# Autodesk Inventor assembly: ASY ДМФ 0100 Барабан v2.1
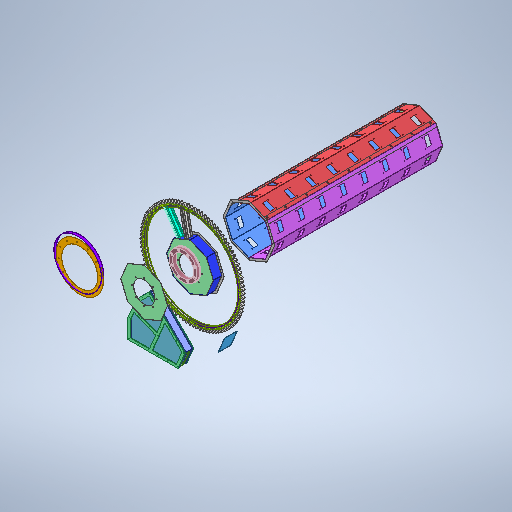
[picture p0: Inventor's stored thumbnail of the model, 512x512]
Saved by Autodesk Inventor 2025 (Build 290162010, 162A)
## iProperties
Created: 2024-04-28
Part Number: ASY ДМФ 0100 Барабан v2.1
Document SubType Name: Assembly
Designer: pokla
Author: pokla
## Documents named in this file (23)
- C:\Users\pokla\Documents\Inventor\ДФО\ДМФ\DMF-Disk-Micro-Filter\Барабан v2.1\ASY ДМФ 0100 Барабан v2.1.iam
- C:\Users\pokla\Documents\Inventor\ДФО\ДМФ\DMF-Disk-Micro-Filter\Барабан v2.1\DMF 01 21 Барабан торец НОС v2.1.ipt
- C:\Users\pokla\Documents\Inventor\ДФО\ДМФ\DMF-Disk-Micro-Filter\Барабан v2.1\DMF 01 13 Барабан Лист лев брт v2.1.ipt
- C:\Users\pokla\Documents\Inventor\ДФО\ДМФ\DMF-Disk-Micro-Filter\Барабан v2.1\DMF 01 14 Барабан Лист прав брт v2.1.ipt
- C:\Users\pokla\Documents\Inventor\ДФО\ДМФ\DMF-Disk-Micro-Filter\Барабан v2.1\DMF 01 31 Барабан Опорное кольцо НОС v2.1.ipt
- C:\Users\pokla\Documents\Inventor\ДФО\ДМФ\DMF-Disk-Micro-Filter\Барабан v2.1\DMF 01 17 опора крышки v2.1.ipt
- C:\Users\pokla\Documents\Inventor\ДФО\ДМФ\DMF-Disk-Micro-Filter\Барабан v2.1\DMF 000 размеры v2.1.ipt
- C:\Users\pokla\Documents\Inventor\ДФО\ДМФ\DMF-Disk-Micro-Filter\Барабан v2.1\DMF 01 12 Барабан усилитель v2.1.ipt
- C:\Users\pokla\Documents\Inventor\ДФО\ДМФ\DMF-Disk-Micro-Filter\Барабан v2.1\ASY DMF 010 cap v2.1.iam
- C:\Users\pokla\Documents\Inventor\ДФО\ДМФ\DMF-Disk-Micro-Filter\Барабан v2.1\DMF 01 32 Барабан Опорное кольцо КОРМА v2.1.ipt
- C:\Users\pokla\Documents\Inventor\ДФО\ДМФ\DMF-Disk-Micro-Filter\Барабан v2.1\DMF 01 22 Барабан торец КОРМА v2.1.ipt
- C:\Users\pokla\Documents\Inventor\ДФО\ДМФ\DMF-Disk-Micro-Filter\Барабан v2.1\ASY DMF filter package v2.1.iam
- C:\Users\pokla\Documents\Inventor\ДФО\ДМФ\DMF-Disk-Micro-Filter\Барабан v2.1\DMF 01 21 cylinder butt end nose.ipt
- C:\Users\pokla\Documents\Inventor\ДФО\ДМФ\DMF-Disk-Micro-Filter\Барабан v2.1\DMF 2.1 01 42 Gear way 2.ipt
- C:\Users\pokla\Documents\Inventor\ДФО\ДМФ\DMF-Disk-Micro-Filter\Барабан v2.1\DMF 2.1 01 43 Gear rim 3.ipt
- C:\Users\pokla\Documents\Inventor\ДФО\ДМФ\DMF-Disk-Micro-Filter\Барабан v2.1\DMF 2.1 01 44 Gear rim 4.ipt
- C:\Users\pokla\Documents\Inventor\ДФО\ДМФ\DMF-Disk-Micro-Filter\Барабан v2.1\DMF 2.1 01 45 Gear ring 5.ipt
- C:\Users\pokla\Documents\Inventor\ДФО\ДМФ\DMF-Disk-Micro-Filter\Барабан v2.1\DMF 2.1 01 46 Gear axis wheel 6.ipt
- C:\Users\pokla\Documents\Inventor\ДФО\ДМФ\DMF-Disk-Micro-Filter\Барабан v2.1\DMF 01 13 Барабан усилитель v2.1.ipt
- C:\Users\pokla\Documents\Inventor\ДФО\ДМФ\DMF-Disk-Micro-Filter\шестерни 06.09.2025\DMF sector big gear 2.1.ipt
- C:\Users\pokla\Documents\Inventor\ДФО\ДМФ\DMF-Disk-Micro-Filter\Барабан v2.1\DMF 01 15 drum sheet 1.ipt
- C:\Users\pokla\Documents\Inventor\ДФО\ДМФ\DMF-Disk-Micro-Filter\ДМФ 01 12 Барабан усилитель.ipt
- C:\Users\pokla\Documents\Inventor\ДФО\ДМФ\DMF-Disk-Micro-Filter\ДМФ 01 15 Барабан усилитель борта.ipt
## Components (86 placed, 26 different names)
1. DMF 000 размеры v2.1.ipt:1
2. DMF 01 21 Барабан торец НОС v2.1.ipt:1 — Rigid:45, Rigid:46, Flush:21
3. DMF 01 31 Барабан Опорное кольцо НОС v2.1.ipt:1
4. DMF 01 32 Барабан Опорное кольцо КОРМА v2.1.ipt:1 — Rigid:20
5. DMF 01 22 Барабан торец КОРМА v2.1.ipt:1 — Rigid:20, Rigid:51, Rigid:53, Mate:36, Flush:22, Flush:23, Mate:37, Flush:24, Flush:25, Mate:38, Flush:26, Flush:27
6. DMF 01 13 Барабан Лист лев брт v2.1.ipt:1 — Rigid:51
7. DMF 01 14 Барабан Лист прав брт v2.1.ipt:1 — Rigid:53
8. DMF 01 17 опора крышки v2.1.ipt:1 — Mate:37, Flush:24, Flush:25
9. DMF 01 17 опора крышки v2.1.ipt:2 — Mate:36, Flush:22, Flush:23
10. ASY DMF 010 cap v2.1.iam:1 [sub-assembly] — Mate:38, Flush:26, Flush:27, Flush:28, Mate:39, Mate:40
11. ASY DMF filter package v2.1.iam:1 [sub-assembly]
12. DMF 01 21 cylinder butt end nose.ipt:1
13. DMF 2.1 01 45 Gear ring 5.ipt:1
14. DMF 2.1 01 46 Gear axis wheel 6.ipt:1
15. DMF 2.1 01 44 Gear rim 4.ipt:1 — Rigid:39, Rigid:40, Rigid:41
16. DMF 2.1 01 43 Gear rim 3.ipt:2 — Rigid:24, Rigid:35
17. DMF 2.1 01 43 Gear rim 3.ipt:1 — Rigid:24
18. DMF 2.1 01 42 Gear way 2.ipt:1
19. DMF 2.1 01 43 Gear rim 3:3 — Rigid:35, Rigid:36, Rigid:39
20. DMF 2.1 01 43 Gear rim 3:4
21. DMF 2.1 01 43 Gear rim 3:5 — Rigid:36, Rigid:38, Flush:18, Mate:33, Mate:34, Tangent:1
22. DMF 2.1 01 43 Gear rim 3:6 — Rigid:42
23. DMF 2.1 01 43 Gear rim 3:7 — Rigid:38
24. DMF 2.1 01 43 Gear rim 3:8
25. DMF 2.1 01 44 Gear rim 4:2 — Rigid:40
26. DMF 2.1 01 44 Gear rim 4:3 — Rigid:41
27. DMF 01 13 Барабан усилитель v2.1.ipt:1 — Rigid:43, Flush:19
28. DMF 01 12 Барабан усилитель v2.1:50 — Flush:18, Mate:33, Mate:34, Rigid:43, Flush:20, Mate:35, Flush:21
29. ДМФ 01 13 Барабан усилитель v2.0:2 — Tangent:1
30. DMF 01 12 Барабан усилитель v2.1:51 — Flush:19, Flush:20
31. DMF 01 15 drum sheet 1:1 — Rigid:46, Flush:29, Mate:41
32. DMF 01 15 drum sheet 1:2 — Rigid:45, Mate:35, Mate:42
33. ДМФ 01 12 Барабан усилитель:1 — Flush:28, Mate:39, Mate:40, Rigid:54, Rigid:55
34. ДМФ 01 15 Барабан усилитель борта:1 — Rigid:54
35. ДМФ 01 15 Барабан усилитель борта:2 — Rigid:55
36. ДМФ 01 12 Барабан усилитель:2 — Flush:29, Mate:41, Mate:42, Rigid:56, Rigid:57
37. ДМФ 01 15 Барабан усилитель борта:3 — Rigid:56
38. ДМФ 01 15 Барабан усилитель борта:4 — Rigid:57
39. DMF sector big gear 2.1.ipt:1 — Rigid:42
40. DMF sector big gear 2.1:2
41. DMF sector big gear 2.1:3
42. DMF sector big gear 2.1:4
43. DMF sector big gear 2.1:5
44. DMF sector big gear 2.1:6
45. DMF sector big gear 2.1:7
46. DMF sector big gear 2.1:8
47. DMF sector big gear 2.1:9
48. DMF sector big gear 2.1:10
49. DMF sector big gear 2.1:11
50. DMF sector big gear 2.1:12
51. DMF sector big gear 2.1:13
52. DMF sector big gear 2.1:14
53. DMF sector big gear 2.1:15
54. DMF sector big gear 2.1:16
55. DMF sector big gear 2.1:17
56. DMF sector big gear 2.1:18
57. DMF sector big gear 2.1:19
58. DMF sector big gear 2.1:20
59. DMF sector big gear 2.1:21
60. DMF sector big gear 2.1:22
61. DMF sector big gear 2.1:23
62. DMF sector big gear 2.1:24
63. DMF sector big gear 2.1:25
64. DMF sector big gear 2.1:26
65. DMF sector big gear 2.1:27
66. DMF sector big gear 2.1:28
67. DMF sector big gear 2.1:29
68. DMF sector big gear 2.1:30
69. DMF sector big gear 2.1:31
70. DMF sector big gear 2.1:32
71. DMF sector big gear 2.1:33
72. DMF sector big gear 2.1:34
73. DMF sector big gear 2.1:35
74. DMF sector big gear 2.1:36
75. DMF sector big gear 2.1:37
76. DMF sector big gear 2.1:38
77. DMF sector big gear 2.1:39
78. DMF sector big gear 2.1:40
79. DMF sector big gear 2.1:41
80. DMF sector big gear 2.1:42
81. DMF sector big gear 2.1:43
82. DMF sector big gear 2.1:44
83. DMF sector big gear 2.1:45
84. DMF sector big gear 2.1:46
85. DMF sector big gear 2.1:47
86. DMF sector big gear 2.1:48
## Component patterns: (48 elements, first: DMF sector big gear 2.1.ipt:1)
## Relationships (45: WeldJoint 22, Flush 12, Mate 10, Tangent 1)
- Rigid:20 [WeldJoint]: DMF 01 32 Барабан Опорное кольцо КОРМА v2.1.ipt:1 ↔ DMF 01 22 Барабан торец КОРМА v2.1.ipt:1
- Rigid:24 [WeldJoint] (25 mm): DMF 2.1 01 43 Gear rim 3.ipt:2 ↔ DMF 2.1 01 43 Gear rim 3.ipt:1
- [WeldJoint] (25 mm): DMF 2.1 01 43 Gear rim 3:3 ↔ DMF 2.1 01 43 Gear rim 3:4
- [WeldJoint] (25 mm): DMF 2.1 01 43 Gear rim 3:5 ↔ DMF 2.1 01 43 Gear rim 3:6
- Rigid:35 [WeldJoint]: DMF 2.1 01 43 Gear rim 3.ipt:2 ↔ DMF 2.1 01 43 Gear rim 3:3
- Rigid:36 [WeldJoint]: DMF 2.1 01 43 Gear rim 3:3 ↔ DMF 2.1 01 43 Gear rim 3:5
- [WeldJoint] (25 mm): DMF 2.1 01 43 Gear rim 3:7 ↔ DMF 2.1 01 43 Gear rim 3:8
- Rigid:38 [WeldJoint]: DMF 2.1 01 43 Gear rim 3:5 ↔ DMF 2.1 01 43 Gear rim 3:7
- Rigid:39 [WeldJoint]: DMF 2.1 01 44 Gear rim 4.ipt:1 ↔ DMF 2.1 01 43 Gear rim 3:3
- Rigid:40 [WeldJoint]: DMF 2.1 01 44 Gear rim 4.ipt:1 ↔ DMF 2.1 01 44 Gear rim 4:2
- Rigid:41 [WeldJoint]: DMF 2.1 01 44 Gear rim 4.ipt:1 ↔ DMF 2.1 01 44 Gear rim 4:3
- Rigid:42 [WeldJoint]: DMF 2.1 01 43 Gear rim 3:6 ↔ DMF sector big gear 2.1.ipt:1
- Flush:18: DMF 2.1 01 43 Gear rim 3:5 ↔ DMF 01 12 Барабан усилитель v2.1:50
- Mate:33: DMF 2.1 01 43 Gear rim 3:5 ↔ DMF 01 12 Барабан усилитель v2.1:50
- Mate:34: DMF 2.1 01 43 Gear rim 3:5 ↔ DMF 01 12 Барабан усилитель v2.1:50
- Rigid:43 [WeldJoint]: DMF 01 13 Барабан усилитель v2.1.ipt:1 ↔ DMF 01 12 Барабан усилитель v2.1:50
- [WeldJoint]: ДМФ 01 13 Барабан усилитель v2.0:2 ↔ DMF 01 12 Барабан усилитель v2.1:51
- Flush:19: DMF 01 13 Барабан усилитель v2.1.ipt:1 ↔ DMF 01 12 Барабан усилитель v2.1:51
- Flush:20: DMF 01 12 Барабан усилитель v2.1:50 ↔ DMF 01 12 Барабан усилитель v2.1:51
- Tangent:1: DMF 2.1 01 43 Gear rim 3:5 ↔ ДМФ 01 13 Барабан усилитель v2.0:2
- Rigid:45 [WeldJoint]: DMF 01 21 Барабан торец НОС v2.1.ipt:1 ↔ DMF 01 15 drum sheet 1:2
- Rigid:46 [WeldJoint]: DMF 01 21 Барабан торец НОС v2.1.ipt:1 ↔ DMF 01 15 drum sheet 1:1
- Mate:35: DMF 01 12 Барабан усилитель v2.1:50 ↔ DMF 01 15 drum sheet 1:2
- Flush:21 (10 mm): DMF 01 21 Барабан торец НОС v2.1.ipt:1 ↔ DMF 01 12 Барабан усилитель v2.1:50
- Rigid:51 [WeldJoint]: DMF 01 22 Барабан торец КОРМА v2.1.ipt:1 ↔ DMF 01 13 Барабан Лист лев брт v2.1.ipt:1
- Rigid:53 [WeldJoint]: DMF 01 22 Барабан торец КОРМА v2.1.ipt:1 ↔ DMF 01 14 Барабан Лист прав брт v2.1.ipt:1
- Mate:36: DMF 01 22 Барабан торец КОРМА v2.1.ipt:1 ↔ DMF 01 17 опора крышки v2.1.ipt:2
- Flush:22 (2 mm): DMF 01 22 Барабан торец КОРМА v2.1.ipt:1 ↔ DMF 01 17 опора крышки v2.1.ipt:2
- Flush:23 (2 mm): DMF 01 22 Барабан торец КОРМА v2.1.ipt:1 ↔ DMF 01 17 опора крышки v2.1.ipt:2
- Mate:37: DMF 01 22 Барабан торец КОРМА v2.1.ipt:1 ↔ DMF 01 17 опора крышки v2.1.ipt:1
- Flush:24 (2 mm): DMF 01 22 Барабан торец КОРМА v2.1.ipt:1 ↔ DMF 01 17 опора крышки v2.1.ipt:1
- Flush:25 (2 mm): DMF 01 22 Барабан торец КОРМА v2.1.ipt:1 ↔ DMF 01 17 опора крышки v2.1.ipt:1
- Mate:38: DMF 01 22 Барабан торец КОРМА v2.1.ipt:1 ↔ ASY DMF 010 cap v2.1.iam:1
- Flush:26: DMF 01 22 Барабан торец КОРМА v2.1.ipt:1 ↔ ASY DMF 010 cap v2.1.iam:1
- Flush:27: DMF 01 22 Барабан торец КОРМА v2.1.ipt:1 ↔ ASY DMF 010 cap v2.1.iam:1
- Flush:28: ASY DMF 010 cap v2.1.iam:1 ↔ ДМФ 01 12 Барабан усилитель:1
- Mate:39: ASY DMF 010 cap v2.1.iam:1 ↔ ДМФ 01 12 Барабан усилитель:1
- Mate:40: ASY DMF 010 cap v2.1.iam:1 ↔ ДМФ 01 12 Барабан усилитель:1
- Rigid:54 [WeldJoint]: ДМФ 01 12 Барабан усилитель:1 ↔ ДМФ 01 15 Барабан усилитель борта:1
- Rigid:55 [WeldJoint]: ДМФ 01 12 Барабан усилитель:1 ↔ ДМФ 01 15 Барабан усилитель борта:2
- Flush:29: DMF 01 15 drum sheet 1:1 ↔ ДМФ 01 12 Барабан усилитель:2
- Mate:41: DMF 01 15 drum sheet 1:1 ↔ ДМФ 01 12 Барабан усилитель:2
- Mate:42: DMF 01 15 drum sheet 1:2 ↔ ДМФ 01 12 Барабан усилитель:2
- Rigid:56 [WeldJoint]: ДМФ 01 12 Барабан усилитель:2 ↔ ДМФ 01 15 Барабан усилитель борта:3
- Rigid:57 [WeldJoint]: ДМФ 01 12 Барабан усилитель:2 ↔ ДМФ 01 15 Барабан усилитель борта:4
## Named parameters: d314_d251 = 25 mm, d315_d251 = 25 mm, d318_d251 = 25 mm, d336_d335 = 0 mm
